# Autodesk Inventor assembly: Tarcza
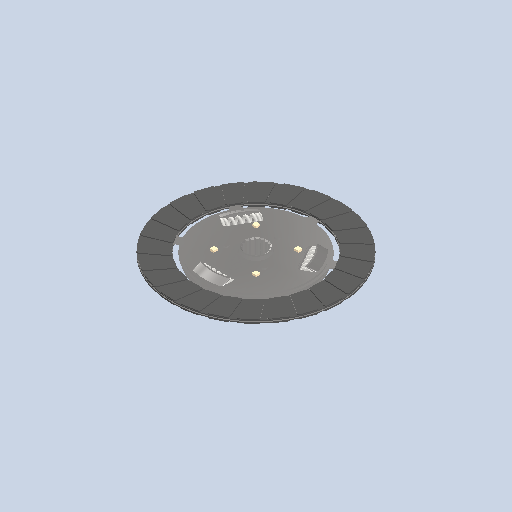
[picture p0: Inventor's stored thumbnail of the model, 512x512]
Saved by Autodesk Inventor 2022 (Build 260153000, 153)
## iProperties
Created: 2021-06-13
Part Number: Tarcza
Document SubType Name: Assembly
Designer: Matik
Author: Matik
## Documents named in this file (14)
- C:\Users\Mateu\Documents\GitHub\ToyotaStarletClutch\ClutchDrivePlate.iam
- C:\Users\Mateu\Documents\GitHub\ToyotaStarletClutch\ClutchDrivePlate_WheelHub.ipt
- C:\Users\Mateu\Documents\GitHub\ToyotaStarletClutch\ClutchDrivePlate_LocatingPad.ipt
- C:\Users\Mateu\Documents\GitHub\ToyotaStarletClutch\ClutchDrivePlate_SlotWasher.ipt
- C:\Users\Mateu\Documents\GitHub\ToyotaStarletClutch\ClutchDrivePlate_FrictionPlate.ipt
- C:\Users\Mateu\Documents\GitHub\ToyotaStarletClutch\ClutchDrivePlate_FrictionLiningA.ipt
- C:\Users\Mateu\Desktop\ToyotaStarletClutch\ClutchDrivePlate_CompressSpring1.ipt
- C:\Users\Mateu\Documents\GitHub\ToyotaStarletClutch\ClutchDrivePlate_CompressSpring3.ipt
- C:\Users\Mateu\Desktop\ToyotaStarletClutch\ClutchDrivePlate_CompressSpring2.ipt
- C:\Users\Mateu\Documents\GitHub\ToyotaStarletClutch\ClutchDrivePlate_FrictionLiningB.ipt
- C:\Users\Mateu\Documents\GitHub\ToyotaStarletClutch\ClutchDrivePlate_CoverA.ipt
- C:\Users\Mateu\Documents\GitHub\ToyotaStarletClutch\ClutchDrivePlate_CoverB.ipt
- C:\Users\Mateu\Documents\GitHub\ToyotaStarletClutch\ClutchDrivePlate_RivetLong.ipt
- C:\Users\Mateu\Desktop\Modele\Tarcza\AIP\FEA\dtygzzj35.fres
## Components (14 placed, 12 different names)
1. ClutchDrivePlate_WheelHub:1 — Wstawiające:1, Wstawiające:2, Wstawiające:3, Wstawiające:4, Wstawiające:5, Wstawiające:6
2. ClutchDrivePlate_LocatingPad:1 — Wstawiające:1, Wstawiające:2, Wstawiające:3, Zestawiające:1, Zestawiające:2, Zestawiające:3, Zestawiające:4, Zestawiające:5, Zestawiające:6, Równoległe:3
3. ClutchDrivePlate_SlotWasher:1 — Zestawiające:1, Zestawiające:2, Zestawiające:3, Równoległe:4
4. ClutchDrivePlate_FrictionPlate:1 — Wstawiające:4, Wstawiające:5, Wstawiające:6, Wstawiające:7, Wstawiające:8, Równoległe:1, Równoległe:2
5. ClutchDrivePlate_FrictionLiningA:1 — Wstawiające:7
6. Compress Spring1:1 — Zestawiające:4
7. Compress Spring2:1 — Zestawiające:6
8. Compress Spring3:1 — Zestawiające:5
9. ClutchDrivePlate_FrictionLiningB:1 — Wstawiające:8
10. ClutchDrivePlate_CoverA:1 — Równoległe:1, Równoległe:2, Równoległe:5, Równoległe:6, Wstawiające:9, Wstawiające:10
11. ClutchDrivePlate_CoverB:1 — Równoległe:3, Równoległe:4
12. ClutchDrivePlate_RivetLong:1 — Równoległe:5, Równoległe:6
13. ClutchDrivePlate_RivetLong:2 — Wstawiające:9
14. ClutchDrivePlate_RivetLong:3 — Wstawiające:10
## Relationships (22: Insert 10, Mate 6, Flush 6)
- Wstawiające:1 [Insert]: ClutchDrivePlate_WheelHub:1 ↔ ClutchDrivePlate_LocatingPad:1
- Wstawiające:2 [Insert]: ClutchDrivePlate_WheelHub:1 ↔ ClutchDrivePlate_LocatingPad:1
- Wstawiające:3 [Insert]: ClutchDrivePlate_WheelHub:1 ↔ ClutchDrivePlate_LocatingPad:1
- Zestawiające:1 [Mate]: ClutchDrivePlate_LocatingPad:1 ↔ ClutchDrivePlate_SlotWasher:1
- Zestawiające:2 [Mate]: ClutchDrivePlate_LocatingPad:1 ↔ ClutchDrivePlate_SlotWasher:1
- Zestawiające:3 [Mate]: ClutchDrivePlate_LocatingPad:1 ↔ ClutchDrivePlate_SlotWasher:1
- Wstawiające:4 [Insert]: ClutchDrivePlate_WheelHub:1 ↔ ClutchDrivePlate_FrictionPlate:1
- Wstawiające:5 [Insert]: ClutchDrivePlate_WheelHub:1 ↔ ClutchDrivePlate_FrictionPlate:1
- Wstawiające:6 [Insert]: ClutchDrivePlate_WheelHub:1 ↔ ClutchDrivePlate_FrictionPlate:1
- Zestawiające:4 [Mate]: ClutchDrivePlate_LocatingPad:1 ↔ Compress Spring1:1
- Zestawiające:5 [Mate]: ClutchDrivePlate_LocatingPad:1 ↔ Compress Spring3:1
- Zestawiające:6 [Mate]: ClutchDrivePlate_LocatingPad:1 ↔ Compress Spring2:1
- Wstawiające:7 [Insert]: ClutchDrivePlate_FrictionPlate:1 ↔ ClutchDrivePlate_FrictionLiningA:1
- Wstawiające:8 [Insert]: ClutchDrivePlate_FrictionPlate:1 ↔ ClutchDrivePlate_FrictionLiningB:1
- Równoległe:1 [Flush]: ClutchDrivePlate_FrictionPlate:1 ↔ ClutchDrivePlate_CoverA:1
- Równoległe:2 [Flush]: ClutchDrivePlate_FrictionPlate:1 ↔ ClutchDrivePlate_CoverA:1
- Równoległe:3 [Flush]: ClutchDrivePlate_LocatingPad:1 ↔ ClutchDrivePlate_CoverB:1
- Równoległe:4 [Flush]: ClutchDrivePlate_SlotWasher:1 ↔ ClutchDrivePlate_CoverB:1
- Równoległe:5 [Flush]: ClutchDrivePlate_CoverA:1 ↔ ClutchDrivePlate_RivetLong:1
- Równoległe:6 [Flush]: ClutchDrivePlate_CoverA:1 ↔ ClutchDrivePlate_RivetLong:1
- Wstawiające:9 [Insert]: ClutchDrivePlate_CoverA:1 ↔ ClutchDrivePlate_RivetLong:2
- Wstawiające:10 [Insert]: ClutchDrivePlate_CoverA:1 ↔ ClutchDrivePlate_RivetLong:3
